# Autodesk Inventor assembly: substrate_plate
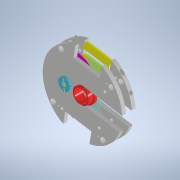
[picture p0: Inventor's stored thumbnail of the model, 180x180]
Saved by Autodesk Inventor 2021 (Build 250183000, 183)
## iProperties
Created: 2024-02-21
Part Number: substrate_plate
Document SubType Name: Assembly
Designer: Sebastián
Author: Sebastián
## Documents named in this file (11)
- C:\Users\Sebastián\Documents\Inventor\PLD SAP\substrate_plate.iam
- C:\Users\Sebastián\Documents\Inventor\PLD SAP\shutter.ipt
- C:\Users\Sebastián\Documents\Inventor\PLD SAP\10d_coupler.ipt
- C:\Users\Sebastián\Documents\Inventor\PLD SAP\muestra.ipt
- C:\Users\Sebastián\Documents\Inventor\PLD SAP\shaft_2.ipt
- C:\Users\Sebastián\Documents\Inventor\PLD SAP\placa_ajuste.iam
- C:\Users\Sebastián\Documents\Inventor\PLD SAP\tape_model.ipt
- C:\Users\Sebastián\Documents\Inventor\PLD SAP\170d_coupler.ipt
- C:\Users\Sebastián\Documents\Inventor\PLD SAP\ang_wedge.ipt
- C:\Users\Sebastián\Documents\Inventor\PLD SAP\5mm_bb.ipt
- C:\Users\Sebastián\Documents\Inventor\PLD SAP\sample_plate.ipt
## Components (13 placed, 10 different names)
1. sample_plate:1 — Angle:1, Rigid:2, Rigid:3, Rigid:4, Rigid:5, Cylindrical:7, Mate:3, Mate:4
2. shutter:1 — Mate:2, Rotational:5
3. 10d_coupler:1 — Rotational:3, Cylindrical:8
4. muestra:1 — Cylindrical:6
5. shaft_2:1 — Rotational:3, Rotational:4, Cylindrical:9
6. placa_ajuste:1 [sub-assembly] — Cylindrical:6, Angle:1, Tangent:1, Tangent:2, Angle:2, Mate:1, Mate:3, Cylindrical:9
7. tape_model:1 — Tangent:1, Tangent:2, Angle:2, Mate:1, Mate:2
8. 170d_coupler:1 — Rotational:4, Cylindrical:7, Mate:4
9. ang_wedge:1 — Rotational:5, Cylindrical:8, Tangent:3
10. 5mm_bb:1 — Rigid:4
11. 5mm_bb:2 — Rigid:2, Tangent:3
12. 5mm_bb:3 — Rigid:5
13. 5mm_bb:4 — Rigid:3
## Relationships (20: CylindricalJoint 4, Mate 4, WeldJoint 4, RevoluteJoint 3, Tangent 3, Angle 2)
- Rotational:3 [RevoluteJoint]: 10d_coupler:1 ↔ shaft_2:1
- Cylindrical:6: muestra:1 ↔ placa_ajuste:1
- Angle:1 (0 deg): sample_plate:1 ↔ placa_ajuste:1
- Tangent:1: placa_ajuste:1 ↔ tape_model:1
- Tangent:2: placa_ajuste:1 ↔ tape_model:1
- Angle:2 (0 deg): placa_ajuste:1 ↔ tape_model:1
- Mate:1 (5 mm): placa_ajuste:1 ↔ tape_model:1
- Mate:2: shutter:1 ↔ tape_model:1
- Rotational:4 [RevoluteJoint]: shaft_2:1 ↔ 170d_coupler:1
- Rigid:2 [WeldJoint]: sample_plate:1 ↔ 5mm_bb:2
- Rigid:3 [WeldJoint]: sample_plate:1 ↔ 5mm_bb:4
- Rigid:4 [WeldJoint]: sample_plate:1 ↔ 5mm_bb:1
- Rigid:5 [WeldJoint]: sample_plate:1 ↔ 5mm_bb:3
- Rotational:5 [RevoluteJoint]: shutter:1 ↔ ang_wedge:1
- Cylindrical:7: sample_plate:1 ↔ 170d_coupler:1
- Mate:3 (11 mm): sample_plate:1 ↔ placa_ajuste:1
- Cylindrical:8: 10d_coupler:1 ↔ ang_wedge:1
- Tangent:3: ang_wedge:1 ↔ 5mm_bb:2
- Mate:4 (1 mm): sample_plate:1 ↔ 170d_coupler:1
- Cylindrical:9: shaft_2:1 ↔ placa_ajuste:1
